# Autodesk Inventor assembly: Camera
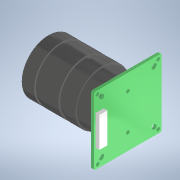
[picture p0: Inventor's stored thumbnail of the model, 180x180]
Saved by Autodesk Inventor 2022 (Build 260153000, 153)
## iProperties
Created: 2022-02-27
Part Number: Camera
Document SubType Name: Assembly
Designer: alexo
Author: alexo
## Documents named in this file (3)
- C:\Users\alexo\Documents\Inventor\Scanner3D\Camera.iam
- C:\Users\alexo\Documents\Inventor\Scanner3D\IMX477_BasisCamera.ipt
- C:\Users\alexo\Documents\Inventor\Scanner3D\IMX477_ElectronicCard.ipt
## Components (2 placed, 2 different names)
1. IMX477_BasisCamera:1 — Rotational:1
2. IMX477_ElectronicCard:1 — Rotational:1
## Relationships (1: RevoluteJoint 1)
- Rotational:1 [RevoluteJoint]: IMX477_BasisCamera:1 ↔ IMX477_ElectronicCard:1
